# Autodesk Inventor assembly: N4049
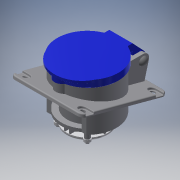
[picture p0: Inventor's stored thumbnail of the model, 180x180]
Saved by Autodesk Inventor 2018 (Build 220112000, 112)
## iProperties
Created: 2021-03-23
Part Number: N4049
Material: Genérico
Document SubType Name: Assembly
Designer: nilton
Author: nilton
## Documents named in this file (7)
- C:\Users\nilto\Dropbox\Tec3GEO\Projetos\Projeto_Sismica\FaseII_Produto\Vibro\Designs\Mecanica\Modelos_3D\Tomadas\N4049.iam
- C:\Users\nilto\Dropbox\Tec3GEO\Projetos\Projeto_Sismica\FaseII_Produto\Vibro\Designs\Mecanica\Modelos_3D\Tomadas\N4049_carcaca.ipt
- C:\Users\nilto\Dropbox\Tec3GEO\Projetos\Projeto_Sismica\FaseII_Produto\Vibro\Designs\Mecanica\Modelos_3D\Tomadas\N4049_tampa_superior.ipt
- C:\Users\nilto\Dropbox\Tec3GEO\Projetos\Projeto_Sismica\FaseII_Produto\Vibro\Designs\Mecanica\Modelos_3D\Tomadas\N4049_pìno_tampa_superior.ipt
- C:\Users\nilto\Dropbox\Tec3GEO\Projetos\Projeto_Sismica\FaseII_Produto\Vibro\Designs\Mecanica\Modelos_3D\Tomadas\N4049_Pino_contato_L.ipt
- C:\Users\nilto\Dropbox\Tec3GEO\Projetos\Projeto_Sismica\FaseII_Produto\Vibro\Designs\Mecanica\Modelos_3D\Tomadas\N4049_pino_contato_T.ipt
- C:\Users\nilto\Dropbox\Tec3GEO\Projetos\Projeto_Sismica\FaseII_Produto\Vibro\Designs\Mecanica\Modelos_3D\Tomadas\N4049_tampa_inferior.ipt
## Components (8 placed, 6 different names)
1. N4049_carcaca:1 — Coincidência:2, Coincidência:3, Coincidência:5, Coincidência:6, Alinhamento:1, Alinhamento:8, Alinhamento:2, Coincidência:7, Coincidência:8, Coincidência:9, Alinhamento:9, Coincidência:10, Coincidência:11, Coincidência:12, Coincidência:13, Alinhamento:10, Ângulo:1
2. N4049_tampa_superior:1 — Coincidência:2, Coincidência:3
3. N4049_pìno_tampa_superior:1 — Coincidência:5, Coincidência:6
4. N4049_Pino_contato_L:1 — Alinhamento:2, Coincidência:9
5. N4049_Pino_contato_L:2 — Alinhamento:8, Coincidência:7
6. N4049_Pino_contato_L:3 — Alinhamento:1, Coincidência:8
7. N4049_pino_contato_T:1 — Alinhamento:9, Coincidência:10
8. N4049_tampa_inferior:1 — Coincidência:11, Coincidência:12, Coincidência:13
## Relationships (17: Mate 11, Flush 5, Angle 1)
- Coincidência:2 [Mate]: N4049_carcaca:1 ↔ N4049_tampa_superior:1
- Coincidência:3 [Mate]: N4049_carcaca:1 ↔ N4049_tampa_superior:1
- Coincidência:5 [Mate]: N4049_carcaca:1 ↔ N4049_pìno_tampa_superior:1
- Coincidência:6 [Mate]: N4049_carcaca:1 ↔ N4049_pìno_tampa_superior:1
- Alinhamento:1 [Flush]: N4049_carcaca:1 ↔ N4049_Pino_contato_L:3
- Alinhamento:8 [Flush]: N4049_carcaca:1 ↔ N4049_Pino_contato_L:2
- Alinhamento:2 [Flush]: N4049_carcaca:1 ↔ N4049_Pino_contato_L:1
- Coincidência:7 [Mate]: N4049_carcaca:1 ↔ N4049_Pino_contato_L:2
- Coincidência:8 [Mate]: N4049_carcaca:1 ↔ N4049_Pino_contato_L:3
- Coincidência:9 [Mate]: N4049_carcaca:1 ↔ N4049_Pino_contato_L:1
- Alinhamento:9 [Flush]: N4049_carcaca:1 ↔ N4049_pino_contato_T:1
- Coincidência:10 [Mate]: N4049_carcaca:1 ↔ N4049_pino_contato_T:1
- Coincidência:11 [Mate]: N4049_carcaca:1 ↔ N4049_tampa_inferior:1
- Coincidência:12 [Mate]: N4049_carcaca:1 ↔ N4049_tampa_inferior:1
- Coincidência:13 [Mate]: N4049_carcaca:1 ↔ N4049_tampa_inferior:1
- Alinhamento:10 [Flush]: N4049_carcaca:1
- Ângulo:1 [Angle] (90 deg): N4049_carcaca:1
